# Autodesk Inventor assembly: Lightswitch
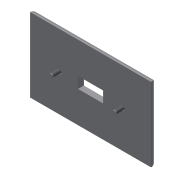
[picture p0: Inventor's stored thumbnail of the model, 180x180]
Saved by Autodesk Inventor 2019 (Build 230136000, 136)
## iProperties
Created: 2019-02-03
Part Number: Lightswitch
Document SubType Name: Assembly
Designer: Jared
Author: Jared
## Documents named in this file (3)
- D:\Jared\Documents\GrabCAD\light-switch-v1\Lightswitch.iam
- D:\Jared\Documents\GrabCAD\light-switch-v1\Plate.ipt
- D:\Jared\Documents\GrabCAD\light-switch-v1\Screw.ipt
## Components (3 placed, 2 different names)
1. Plate:1 — Mate:1, Mate:2, Mate:3, Mate:4
2. Screw:1 — Mate:2, Mate:4
3. Screw:2 — Mate:1, Mate:3
## Relationships (4: Mate 4)
- Mate:1: Plate:1 ↔ Screw:2
- Mate:2: Plate:1 ↔ Screw:1
- Mate:3: Plate:1 ↔ Screw:2
- Mate:4: Plate:1 ↔ Screw:1
